# Autodesk Inventor assembly: FirstTryAssembly
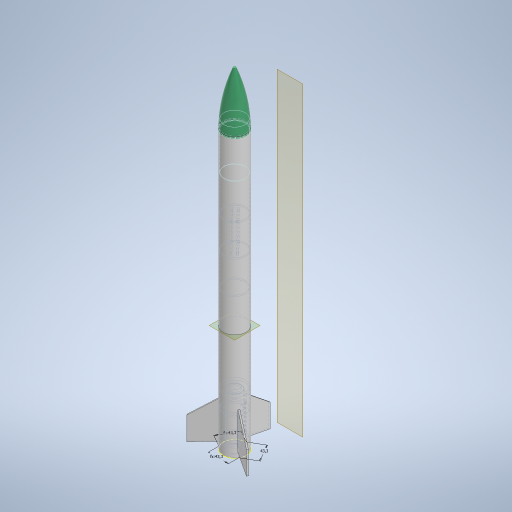
[picture p0: Inventor's stored thumbnail of the model, 512x512]
Saved by Autodesk Inventor 2023.2 (Build 272271000, 271)
## iProperties
Created: 2022-12-18
Part Number: FirstTryAssembly
Document SubType Name: Assembly
Designer: Admin
Author: Admin
## Documents named in this file (9)
- C:\Users\Admin\Desktop\PUT RocketLab\Rakietka\FirstTryAssembly.iam
- C:\Users\Admin\Desktop\PUT RocketLab\Rakietka\Korpus.ipt
- C:\Users\Admin\Desktop\PUT RocketLab\Rakietka\EngineBlock.ipt
- C:\Users\Admin\Desktop\PUT RocketLab\Rakietka\nose-cone.ipt
- C:\Users\Admin\Desktop\PUT RocketLab\Rakietka\PrzegrodaNaElektronike.ipt
- C:\Users\Admin\Desktop\PUT RocketLab\Rakietka\RuraWewnetrznaSilnik.ipt
- C:\Users\Admin\Desktop\PUT RocketLab\Rakietka\Stateczniki.ipt
- C:\Users\Admin\Desktop\PUT RocketLab\Rakietka\CenterRing.ipt
- C:\Users\Admin\Desktop\PUT RocketLab\Rakietka\koszyk na elektro.ipt
## Components (11 placed, 8 different names)
1. Korpus:1 — Mate:3, Mate:4, Mate:5, Mate:6, Mate:7, Mate:8, Flush:2, Mate:9, Flush:3, Mate:12, Mate:13, Flush:6, Mate:14, Mate:15, Mate:16, Mate:17, Mate:18, Mate:19
2. EngineBlock:1 — Mate:7, Flush:1
3. nose-cone:1 — Mate:12, Mate:21
4. RuraWewnetrznaSilnik:1 — Mate:3, Mate:6, Flush:1, Mate:20, Flush:7, Flush:8
5. Stateczniki:1 — Mate:4, Mate:5, Mate:13, Flush:6
6. Stateczniki:2 — Mate:14, Mate:15, Mate:16
7. Stateczniki:3 — Mate:17, Mate:18, Mate:19
8. CenterRing:1 — Mate:9, Flush:3
9. CenterRing:2 — Mate:8, Flush:2
10. koszyk na elektro:1 — Mate:20, Flush:7
11. PrzegrodaNaElektronike:1 — Mate:21, Flush:8
## Relationships (23: Mate 17, Flush 6)
- Mate:3: Korpus:1 ↔ RuraWewnetrznaSilnik:1
- Mate:4: Korpus:1 ↔ Stateczniki:1
- Mate:5: Korpus:1 ↔ Stateczniki:1
- Mate:6: Korpus:1 ↔ RuraWewnetrznaSilnik:1
- Mate:7: Korpus:1 ↔ EngineBlock:1
- Flush:1 (5 mm): EngineBlock:1 ↔ RuraWewnetrznaSilnik:1
- Mate:8: Korpus:1 ↔ CenterRing:2
- Flush:2 (17 mm): Korpus:1 ↔ CenterRing:2
- Mate:9: Korpus:1 ↔ CenterRing:1
- Flush:3 (75 mm): Korpus:1 ↔ CenterRing:1
- Mate:12: Korpus:1 ↔ nose-cone:1
- Mate:13: Korpus:1 ↔ Stateczniki:1
- Flush:6 (-10.5 mm): Korpus:1 ↔ Stateczniki:1
- Mate:14: Korpus:1 ↔ Stateczniki:2
- Mate:15: Korpus:1 ↔ Stateczniki:2
- Mate:16 (25 mm): Korpus:1 ↔ Stateczniki:2
- Mate:17: Korpus:1 ↔ Stateczniki:3
- Mate:18: Korpus:1 ↔ Stateczniki:3
- Mate:19 (25 mm): Korpus:1 ↔ Stateczniki:3
- Mate:20: RuraWewnetrznaSilnik:1 ↔ koszyk na elektro:1
- Flush:7 (370 mm): RuraWewnetrznaSilnik:1 ↔ koszyk na elektro:1
- Mate:21: nose-cone:1 ↔ PrzegrodaNaElektronike:1
- Flush:8 (300 mm): RuraWewnetrznaSilnik:1 ↔ PrzegrodaNaElektronike:1
